# Autodesk Inventor assembly: Banebots RS-775 P60 Planetary Gearbox 4  to 1 (0.5x1.5 shaft)
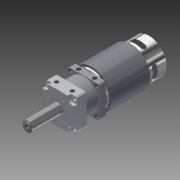
[picture p0: Inventor's stored thumbnail of the model, 180x180]
Saved by Autodesk Inventor 2013 (Build 170138000, 138)
## iProperties
Created: 2013-03-11
Part Number: Banebots RS-775 P60 Planetary Gearbox 4  to 1 (0.5x1.5 shaft)
Document SubType Name: Assembly
Designer: Moses
Mass: 464.754 g
Surface Area: 443.388 cm^2
Volume: 60.4329 cm^3
Density: 7.69042 g/cm^3
Author: Moses
## Documents named in this file (7)
- C:\Users\Moses\Documents\GitHub\frc2013CAD\Drivetrain\Toughbox-mini\Banebots P60\Banebots RS-775 P60 Planetary Gearbox 4  to 1 (0.5x1.5 shaft).iam
- C:\Users\Moses\Documents\GitHub\frc2013CAD\Drivetrain\Toughbox-mini\Banebots P60\Gearbox End Plate.ipt
- C:\Users\Moses\Documents\GitHub\frc2013CAD\Drivetrain\Toughbox-mini\Banebots P60\Gearbox Ring Gear 4 to 1.ipt
- C:\Users\Moses\Documents\GitHub\frc2013CAD\Drivetrain\Toughbox-mini\Banebots P60\Gearbox End Plate 2.ipt
- C:\Users\Moses\Documents\GitHub\frc2013CAD\Drivetrain\Toughbox-mini\Banebots P60\Motors_BaneBots_RS-775.ipt
- C:\Users\Moses\Documents\GitHub\frc2013CAD\Drivetrain\Toughbox-mini\Banebots P60\R6Z Ball Bearing (0.375x0.875).ipt
- C:\Users\Moses\Documents\GitHub\frc2013CAD\Drivetrain\Toughbox-mini\Banebots P60\Banebots 0.5x1.5 P60 Shaft.ipt
## Components (7 placed, 6 different names)
1. Gearbox End Plate:1 — Insert:5, Insert:7, Insert:8
2. Gearbox Ring Gear 4 to 1:1 — Insert:5, Insert:6
3. Gearbox End Plate 2:1 — Insert:6, Insert:10
4. Motors_BaneBots_RS-775:1 — Insert:10
5. R6Z Ball Bearing (0.375x0.875):1 — Insert:8, Insert:9
6. R6Z Ball Bearing (0.375x0.875):2 — Insert:7
7. Banebots 0.5x1.5 P60 Shaft:1 — Insert:9
## Relationships (6: Insert 6)
- Insert:5: Gearbox End Plate:1 ↔ Gearbox Ring Gear 4 to 1:1
- Insert:6: Gearbox Ring Gear 4 to 1:1 ↔ Gearbox End Plate 2:1
- Insert:7: Gearbox End Plate:1 ↔ R6Z Ball Bearing (0.375x0.875):2
- Insert:8: Gearbox End Plate:1 ↔ R6Z Ball Bearing (0.375x0.875):1
- Insert:9: R6Z Ball Bearing (0.375x0.875):1 ↔ Banebots 0.5x1.5 P60 Shaft:1
- Insert:10: Gearbox End Plate 2:1 ↔ Motors_BaneBots_RS-775:1
